# Autodesk Inventor assembly: 上部分
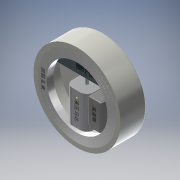
[picture p0: Inventor's stored thumbnail of the model, 180x180]
Saved by Autodesk Inventor 2018.3 (Build 223284000, 284)
## iProperties
Created: 2018-12-27
Part Number: 上部分
Material: 常规
Document SubType Name: Assembly
Designer: 丁子鸣
Author: 丁子鸣
## Documents named in this file (7)
- C:\Users\丁子鸣\Desktop\比赛图\上部分.iam
- C:\Users\丁子鸣\Desktop\比赛图\上盖板.ipt
- C:\Users\丁子鸣\Desktop\比赛图\配重.ipt
- C:\Users\丁子鸣\Desktop\比赛图\轴承外圈.ipt
- C:\Users\丁子鸣\Desktop\比赛图\轴承内圈.ipt
- C:\Users\丁子鸣\Desktop\比赛图\液压马达.ipt
- C:\Users\丁子鸣\Desktop\比赛图\减速箱.ipt
## Components (6 placed, 6 different names)
1. 上盖板:1 — 配合:1, 配合:2, 表面齐平:1, 配合:3, 表面齐平:3, 表面齐平:4
2. 配重:1 — 配合:1, 配合:2, 配合:5, 配合:6
3. 轴承外圈:1 — 表面齐平:1, 配合:3, 表面齐平:2, 配合:4
4. 轴承内圈:1 — 表面齐平:2, 配合:4
5. 液压马达:1 — 表面齐平:3, 配合:5
6. 减速箱:1 — 表面齐平:4, 配合:6
## Relationships (10: Mate 6, Flush 4)
- 配合:1 [Mate]: 上盖板:1 ↔ 配重:1
- 配合:2 [Mate]: 上盖板:1 ↔ 配重:1
- 表面齐平:1 [Flush]: 上盖板:1 ↔ 轴承外圈:1
- 配合:3 [Mate]: 上盖板:1 ↔ 轴承外圈:1
- 表面齐平:2 [Flush]: 轴承外圈:1 ↔ 轴承内圈:1
- 配合:4 [Mate]: 轴承外圈:1 ↔ 轴承内圈:1
- 表面齐平:3 [Flush]: 上盖板:1 ↔ 液压马达:1
- 表面齐平:4 [Flush]: 上盖板:1 ↔ 减速箱:1
- 配合:5 [Mate] (80 mm): 配重:1 ↔ 液压马达:1
- 配合:6 [Mate] (75 mm): 配重:1 ↔ 减速箱:1
